# Autodesk Inventor assembly: DiscoDraw
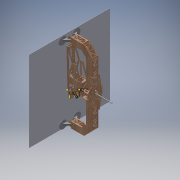
[picture p0: Inventor's stored thumbnail of the model, 180x180]
Saved by Autodesk Inventor 2019 (Build 230136000, 136)
## iProperties
Created: 2019-01-14
Part Number: DiscoDraw
Document SubType Name: Assembly
Designer: nxgam
Author: nxgam
## Documents named in this file (4)
- C:\Users\nxgam\Documents\CAD\Inventor\DiscoDraw\DiscoDraw.iam
- C:\Users\nxgam\Documents\CAD\Inventor\DiscoDraw\Gantry.iam
- C:\Users\nxgam\Documents\CAD\Inventor\DiscoDraw\Arm.iam
- C:\Users\nxgam\Documents\CAD\Inventor\DiscoDraw\White Board.ipt
## Components (3 placed, 3 different names)
1. Gantry:1 [sub-assembly] — Mate:1, Mate:2
2. Arm:1 [sub-assembly] — Mate:1
3. White Board:1 — Mate:2, Mate:3, Mate:4
## Relationships (4: Mate 4)
- Mate:1: Gantry:1 ↔ Arm:1
- Mate:2: Gantry:1 ↔ White Board:1
- Mate:3: White Board:1
- Mate:4: White Board:1
